# Autodesk Inventor assembly: Rb oven housing
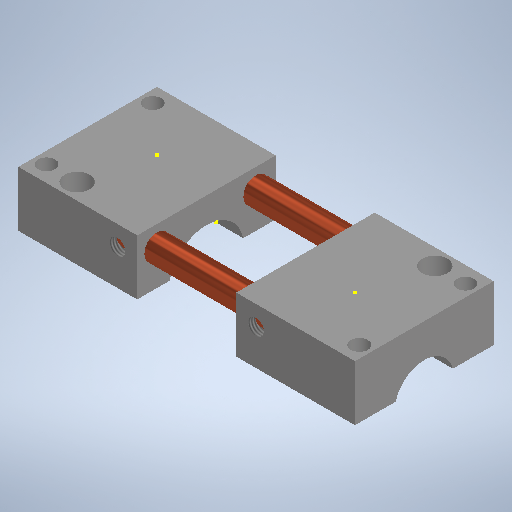
[picture p0: Inventor's stored thumbnail of the model, 512x512]
Saved by Autodesk Inventor 2025.3 (Build 293356000, 356)
## iProperties
Created: 2025-04-24
Part Number: Rb oven housing
Document SubType Name: Assembly
Designer: E. Moreno
Author: E. Moreno
Title: Carcasa Horno - Ensamblado
## Documents named in this file (4)
- E:\Users\USER\Documents\GitHub\LAFriOC\Rb oven\Rb housing\Rb oven housing - Top.iam
- E:\Users\USER\Documents\GitHub\LAFriOC\Rb oven\Rb housing\Rb oven housing post.ipt
- E:\Users\USER\Documents\GitHub\LAFriOC\Rb oven\Rb housing\Rb oven housing top-back_front.ipt
- E:\Users\USER\Documents\GitHub\LAFriOC\Rb oven\Rb housing\Rb oven housing top-back_front_MIR_MIR.ipt
## Components (4 placed, 3 different names)
1. Rb oven housing top-back_front:1 — Insert:1, Insert:2
2. Rb oven housing post:3 — Insert:2
3. Rb oven housing post:4 — Insert:1, Insert:3
4. Rb oven housing top-back_front_MIR_MIR:1 — Insert:3
## Relationships (3: Insert 3)
- Insert:1 (-15 mm): Rb oven housing top-back_front:1 ↔ Rb oven housing post:4
- Insert:2 (-15 mm): Rb oven housing top-back_front:1 ↔ Rb oven housing post:3
- Insert:3 (-15 mm): Rb oven housing post:4 ↔ Rb oven housing top-back_front_MIR_MIR:1
